# Autodesk Inventor assembly: Assembly_Cube_LED_holder_v3
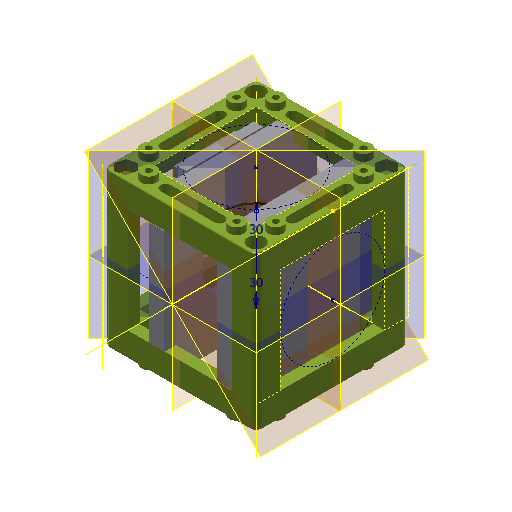
[picture p0: Inventor's stored thumbnail of the model, 512x512]
Saved by Autodesk Inventor 2022 (Build 260153000, 153)
## iProperties
Created: 2019-08-07
Part Number: Assembly_Cube_LED_holder_v3
Document SubType Name: Assembly
Designer: marsikovabarbora
Author: marsikovabarbora
## Documents named in this file (6)
- C:\Users\PrakashLab\Documents\UC2-INVENTOR-Git\uc2_v3\Assembly_Cube_LED_holder_v3.iam
- C:\Users\PrakashLab\Documents\UC2-INVENTOR-Git\uc2_v3\Assembly_Cube_empty_IM_v3.iam
- C:\Users\PrakashLab\Documents\UC2-INVENTOR-Git\uc2_v3\20_Cube_insert_Sample_holder_v3.ipt
- C:\Users\PrakashLab\Documents\UC2-INVENTOR-Git\uc2_v3\20_Cube_Insert_Sample_clamp.ipt
- C:\Users\PrakashLab\Documents\UC2-INVENTOR-Git\uc2_v3\00_3W_LED_Star_pad_v1.iam
- C:\Users\PrakashLab\Documents\UC2-INVENTOR-Git\uc2_v3\20_Cube_insert_LED_holder_v3.ipt
## Components (5 placed, 5 different names)
1. Assembly_Cube_empty_IM_v3:1 [sub-assembly] — Mate:1, Mate:2, Flush:1, Mate:12, Angle:2, Mate:13, Mate:15, Flush:2, Flush:3, Mate:16
2. 20_Cube_insert_LED_holder_v3:1 — Mate:14, Mate:15, Flush:2, Flush:3
3. 00_3W_LED_Star_pad_v1:1 [sub-assembly] — Mate:14, Mate:16
4. 20_Cube_Insert_Sample_clamp:1 — Mate:9, Mate:10, Mate:11
5. 20_Cube_insert_Sample_holder_v3:1 — Mate:9, Mate:10, Mate:11, Mate:12, Angle:2, Mate:13
## Relationships (14: Mate 10, Flush 3, Angle 1)
- Mate:1: Assembly_Cube_empty_IM_v3:1
- Mate:2: Assembly_Cube_empty_IM_v3:1
- Flush:1: Assembly_Cube_empty_IM_v3:1
- Mate:9: 20_Cube_Insert_Sample_clamp:1 ↔ 20_Cube_insert_Sample_holder_v3:1
- Mate:10: 20_Cube_Insert_Sample_clamp:1 ↔ 20_Cube_insert_Sample_holder_v3:1
- Mate:11: 20_Cube_Insert_Sample_clamp:1 ↔ 20_Cube_insert_Sample_holder_v3:1
- Mate:12: Assembly_Cube_empty_IM_v3:1 ↔ 20_Cube_insert_Sample_holder_v3:1
- Angle:2 (0 deg): Assembly_Cube_empty_IM_v3:1 ↔ 20_Cube_insert_Sample_holder_v3:1
- Mate:13: Assembly_Cube_empty_IM_v3:1 ↔ 20_Cube_insert_Sample_holder_v3:1
- Mate:14: 20_Cube_insert_LED_holder_v3:1 ↔ 00_3W_LED_Star_pad_v1:1
- Mate:15: Assembly_Cube_empty_IM_v3:1 ↔ 20_Cube_insert_LED_holder_v3:1
- Flush:2: Assembly_Cube_empty_IM_v3:1 ↔ 20_Cube_insert_LED_holder_v3:1
- Flush:3: Assembly_Cube_empty_IM_v3:1 ↔ 20_Cube_insert_LED_holder_v3:1
- Mate:16: Assembly_Cube_empty_IM_v3:1 ↔ 00_3W_LED_Star_pad_v1:1
